# Autodesk Inventor assembly: table
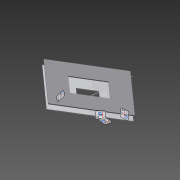
[picture p0: Inventor's stored thumbnail of the model, 180x180]
Saved by Autodesk Inventor 2015 (Build 190159000, 159)
## iProperties
Created: 2019-04-10
Part Number: table
Document SubType Name: Assembly
Designer: Raptor
Author: Raptor
## Documents named in this file (5)
- C:\Users\Raptor\Desktop\table\table.iam
- C:\Users\Raptor\Desktop\table\top long.ipt
- C:\Users\Raptor\Desktop\table\top short.ipt
- C:\Users\Raptor\Desktop\table\bottom long.ipt
- C:\Users\Raptor\Desktop\table\bottom short.ipt
## Components (8 placed, 4 different names)
1. bottom long:1 — Mate:7, Mate:8, Flush:4, Mate:9, Flush:5, Mate:10
2. bottom short:1 — Mate:7, Mate:8, Flush:4, Mate:12, Mate:14
3. bottom short:2 — Mate:9, Flush:5, Mate:10, Mate:11, Flush:6, Flush:9
4. bottom long:2 — Mate:11, Flush:6, Mate:12, Flush:8, Mate:13
5. top short:2 — Mate:5, Flush:3, Mate:6, Flush:9
6. top long:2 — Mate:3, Flush:2, Mate:4, Mate:6
7. top short:1 — Mate:1, Mate:2, Flush:1, Mate:3, Flush:2, Mate:4
8. top long:1 — Mate:1, Mate:2, Flush:1, Mate:5, Flush:3, Flush:8, Mate:13
## Relationships (22: Mate 14, Flush 8)
- Mate:1: top short:1 ↔ top long:1
- Mate:2: top short:1 ↔ top long:1
- Flush:1: top short:1 ↔ top long:1
- Mate:3: top long:2 ↔ top short:1
- Flush:2: top long:2 ↔ top short:1
- Mate:4: top long:2 ↔ top short:1
- Mate:5: top short:2 ↔ top long:1
- Flush:3: top short:2 ↔ top long:1
- Mate:6: top short:2 ↔ top long:2
- Mate:7: bottom long:1 ↔ bottom short:1
- Mate:8: bottom long:1 ↔ bottom short:1
- Flush:4: bottom long:1 ↔ bottom short:1
- Mate:9: bottom long:1 ↔ bottom short:2
- Flush:5: bottom long:1 ↔ bottom short:2
- Mate:10: bottom long:1 ↔ bottom short:2
- Mate:11: bottom short:2 ↔ bottom long:2
- Flush:6: bottom short:2 ↔ bottom long:2
- Mate:12: bottom short:1 ↔ bottom long:2
- Flush:8: bottom long:2 ↔ top long:1
- Flush:9: bottom short:2 ↔ top short:2
- Mate:13 (100 mm): bottom long:2 ↔ top long:1
- Mate:14: bottom short:1
